# Autodesk Inventor assembly: СТУЛЬЧАКИ
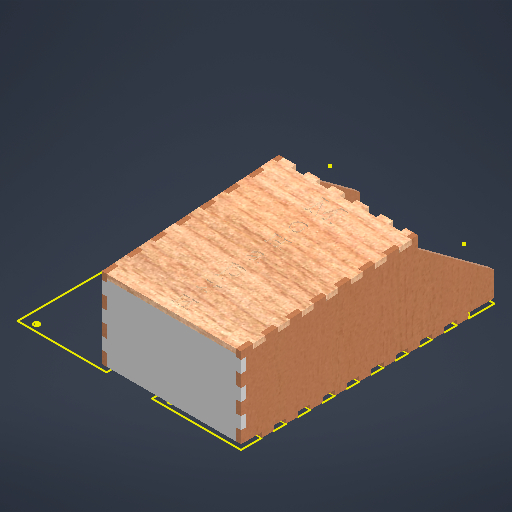
[picture p0: Inventor's stored thumbnail of the model, 512x512]
Saved by Autodesk Inventor 2025 (Build 290162000, 162)
## iProperties
Created: 2025-01-29
Part Number: СТУЛЬЧАКИ
Document SubType Name: Assembly
Designer: Phantom
Author: Phantom
## Documents named in this file (4)
- C:\Users\Phantom\Desktop\Phantom16950\СТУЛЬЧАКИ.iam
- C:\Users\Phantom\Desktop\Phantom16950\стульчак 2.ipt
- C:\Users\Phantom\Desktop\Phantom16950\стульчак 3.ipt
- C:\Users\Phantom\Desktop\Phantom16950\стульчак 4.ipt
## Components (4 placed, 3 different names)
1. стульчак 2:1 — Заподлицо:1, Заподлицо:2, Совмещение:2
2. стульчак 3:1 — Совмещение:1
3. стульчак 2:2 — Совмещение:1, Заподлицо:1, Заподлицо:2, Заподлицо:3, Заподлицо:4
4. стульчак 4:1 — Заподлицо:3, Заподлицо:4, Совмещение:2
## Relationships (6: Flush 4, Mate 2)
- Совмещение:1 [Mate]: стульчак 3:1 ↔ стульчак 2:2
- Заподлицо:1 [Flush]: стульчак 2:1 ↔ стульчак 2:2
- Заподлицо:2 [Flush]: стульчак 2:1 ↔ стульчак 2:2
- Заподлицо:3 [Flush]: стульчак 2:2 ↔ стульчак 4:1
- Заподлицо:4 [Flush]: стульчак 2:2 ↔ стульчак 4:1
- Совмещение:2 [Mate]: стульчак 2:1 ↔ стульчак 4:1
